# Autodesk Inventor assembly: ToggleSwitch_SPST_13x7
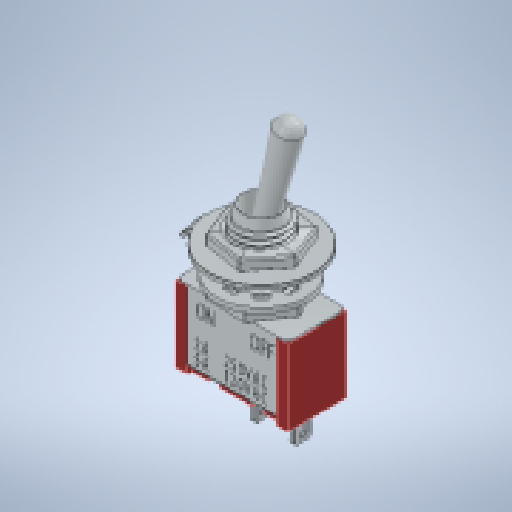
[picture p0: Inventor's stored thumbnail of the model, 512x512]
Saved by Autodesk Inventor 2025.1 (Build 291241020, 241B)
## iProperties
Created: 2024-11-08
Part Number: ToggleSwitch_SPST_13x7
Document SubType Name: Assembly
Designer: leon-
Sending System: SolidWorks 2023
Last Author: Don
Last Saved: 2024-11-11
Author: leon-
## Documents named in this file (8)
- C:\Users\leon-\OneDrive\Dokumente\Education\Berkeley\Embedded_Systems\Project\MagDrop4\CAD_Model\Purchase_Parts\Electronics\On-Off_Switch\ToggleSwitch_SPST_13x7.iam
- C:\Users\leon-\OneDrive\Dokumente\Education\Berkeley\Embedded_Systems\Project\MagDrop4\CAD_Model\Purchase_Parts\Electronics\On-Off_Switch\ToggleSwitch_SPST_Base.ipt
- C:\Users\leon-\OneDrive\Dokumente\Education\Berkeley\Embedded_Systems\Project\MagDrop4\CAD_Model\Purchase_Parts\Electronics\On-Off_Switch\ToggleSwitch_SPST_BaseCove.ipt
- C:\Users\leon-\OneDrive\Dokumente\Education\Berkeley\Embedded_Systems\Project\MagDrop4\CAD_Model\Purchase_Parts\Electronics\On-Off_Switch\ToggleSwitch_SPST_Lever.ipt
- C:\Users\leon-\OneDrive\Dokumente\Education\Berkeley\Embedded_Systems\Project\MagDrop4\CAD_Model\Purchase_Parts\Electronics\On-Off_Switch\ToggleSwitch_SPST_Washer_T.ipt
- C:\Users\leon-\OneDrive\Dokumente\Education\Berkeley\Embedded_Systems\Project\MagDrop4\CAD_Model\Purchase_Parts\Electronics\On-Off_Switch\ToggleSwitch_SPST_Washer_S.ipt
- C:\Users\leon-\OneDrive\Dokumente\Education\Berkeley\Embedded_Systems\Project\MagDrop4\CAD_Model\Purchase_Parts\Electronics\On-Off_Switch\ToggleSwitch_SPST_Terminal.ipt
- C:\Users\leon-\OneDrive\Dokumente\Education\Berkeley\Embedded_Systems\Project\MagDrop4\CAD_Model\Purchase_Parts\Electronics\On-Off_Switch\ToggleSwitch_SPST_Nut_Side.ipt
## Components (9 placed, 7 different names)
1. ToggleSwitch_SPST_Base:1
2. ToggleSwitch_SPST_BaseCover:1 — Mate:1, Mate:2
3. ToggleSwitch_SPST_Lever:1
4. ToggleSwitch_SPST_Washer_Toothed:1
5. ToggleSwitch_SPST_Washer_SingleKey:1 — Mate:1, Mate:3
6. ToggleSwitch_SPST_Terminal:1
7. ToggleSwitch_SPST_Terminal:2
8. ToggleSwitch_SPST_Nut_Sided:1 — Mate:2, Mate:3
9. ToggleSwitch_SPST_Nut_Sided:2
## Relationships (3: Mate 3)
- Mate:1: ToggleSwitch_SPST_BaseCover:1 ↔ ToggleSwitch_SPST_Washer_SingleKey:1
- Mate:2: ToggleSwitch_SPST_BaseCover:1 ↔ ToggleSwitch_SPST_Nut_Sided:1
- Mate:3: ToggleSwitch_SPST_Washer_SingleKey:1 ↔ ToggleSwitch_SPST_Nut_Sided:1
